# Autodesk Inventor assembly: Assembly1
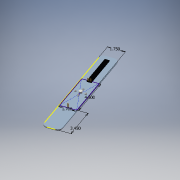
[picture p0: Inventor's stored thumbnail of the model, 180x180]
Saved by Autodesk Inventor 2016 (Build 200138000, 138)
## iProperties
Created: 2017-12-11
Part Number: Assembly1
Document SubType Name: Assembly
Designer: student
Author: student
## Documents named in this file (4)
- C:\Users\student\Documents\GitHub\POV2017\INVENTOR\Assembly1.iam
- C:\Users\student\Documents\GitHub\POV2017\INVENTOR\Base.ipt
- C:\Users\student\Documents\GitHub\POV2017\INVENTOR\Shaft.ipt
- C:\Users\student\Documents\Inventor\Content Center Files\R2016\en-US\GB 6560-86\Screw GB 6560-86 M3 x 6.ipt
## Components (6 placed, 3 different names)
1. Base:1 — Mate:2, Mate:3, Mate:4, Insert:1, Insert:2, Insert:3, Insert:4
2. Shaft:1 — Mate:2, Mate:3, Mate:4
3. Tapping screw GB/T 6560-1986 M3x6:1 — Insert:1
4. Tapping screw GB/T 6560-1986 M3x6:2 — Insert:2
5. Tapping screw GB/T 6560-1986 M3x6:3 — Insert:3
6. Tapping screw GB/T 6560-1986 M3x6:4 — Insert:4
## Relationships (7: Insert 4, Mate 3)
- Mate:2: Base:1 ↔ Shaft:1
- Mate:3: Base:1 ↔ Shaft:1
- Mate:4: Base:1 ↔ Shaft:1
- Insert:1: Base:1 ↔ Tapping screw GB/T 6560-1986 M3x6:1
- Insert:2: Base:1 ↔ Tapping screw GB/T 6560-1986 M3x6:2
- Insert:3: Base:1 ↔ Tapping screw GB/T 6560-1986 M3x6:3
- Insert:4: Base:1 ↔ Tapping screw GB/T 6560-1986 M3x6:4
